# Autodesk Inventor assembly: Assembly1
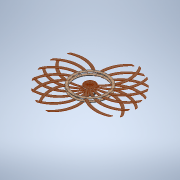
[picture p0: Inventor's stored thumbnail of the model, 180x180]
Saved by Autodesk Inventor 2020.3 (Build 243373000, 373)
## iProperties
Created: 2020-11-01
Part Number: Assembly1
Document SubType Name: Assembly
Designer: Martijn
Author: Martijn
## Documents named in this file (28)
- D:\Documents\GitHub\electrokinetic-sculpture\cad files\Assembly1.iam
- D:\Documents\GitHub\electrokinetic-sculpture\cad files\as.ipt
- D:\Documents\GitHub\electrokinetic-sculpture\cad files\pulley1.ipt
- D:\Documents\GitHub\electrokinetic-sculpture\cad files\wall_mount.ipt
- D:\Documents\GitHub\electrokinetic-sculpture\cad files\GT2 60 teeth pulley.ipt
- D:\Documents\GitHub\electrokinetic-sculpture\cad files\Nema 17 - Busheng 17HD34008-22B\Nema 17 Stepper Motor.iam
- D:\Documents\GitHub\electrokinetic-sculpture\cad files\bearing_holder.ipt
- D:\Documents\GitHub\electrokinetic-sculpture\cad files\bearing_holder2.ipt
- D:\Documents\GitHub\electrokinetic-sculpture\cad files\enclosure.ipt
- D:\Documents\GitHub\electrokinetic-sculpture\cad files\Lock Collar 8mm.ipt
- D:\Documents\GitHub\electrokinetic-sculpture\cad files\spoke.ipt
- D:\Documents\GitHub\electrokinetic-sculpture\cad files\spoke2.ipt
- D:\Documents\GitHub\electrokinetic-sculpture\cad files\cover.ipt
- D:\Documents\GitHub\electrokinetic-sculpture\cad files\pololu-universal-aluminum-mounting-hub-for-8mm-shaft-m3-holes.ipt
- D:\Documents\GitHub\electrokinetic-sculpture\cad files\wheel2.ipt
- D:\Documents\GitHub\electrokinetic-sculpture\cad files\front_plate.ipt
- D:\Documents\GitHub\electrokinetic-sculpture\cad files\spoke3.ipt
- D:\Documents\GitHub\electrokinetic-sculpture\cad files\cover2.ipt
- D:\Documents\GitHub\electrokinetic-sculpture\cad files\wheel3.ipt
- D:\Documents\GitHub\electrokinetic-sculpture\cad files\wheel4.ipt
- D:\Documents\GitHub\electrokinetic-sculpture\cad files\spoke4.ipt
- D:\Documents\GitHub\electrokinetic-sculpture\cad files\wheel5.ipt
- D:\Documents\GitHub\electrokinetic-sculpture\cad files\wheel6.ipt
- D:\Documents\GitHub\electrokinetic-sculpture\cad files\wheel7.ipt
- D:\Documents\GitHub\electrokinetic-sculpture\cad files\wheel8.ipt
- D:\Documents\GitHub\electrokinetic-sculpture\cad files\center_cover.ipt
- D:\Documents\GitHub\electrokinetic-sculpture\cad files\motor_spacer.ipt
- D:\Documents\GitHub\electrokinetic-sculpture\cad files\pulley_bearing_combo.ipt
## Components (72 placed, 27 different names)
1. as:1 — Mate:2, Flush:1, Mate:13, Mate:20, Mate:64, Mate:213, Mate:260, Mate:262, Mate:264
2. pulley1:1 — Mate:22, Mate:24, Mate:27, Mate:30, Mate:33, Mate:61, Mate:63, Mate:66, Mate:212, Mate:213, Mate:214, Mate:215, Mate:216, Mate:217, Mate:218, Mate:219, Mate:220, Mate:221, Mate:222, Mate:223, Mate:224, Mate:225, Mate:226, Mate:227, Mate:228, Mate:229, Mate:230, Mate:231, Mate:232, Mate:233, Mate:234, Mate:235, Mate:236, Mate:237, Mate:238, Mate:239, Mate:240, Mate:241, Mate:242, Mate:244, Mate:245, Mate:246, Mate:247, Mate:248, Mate:249, Mate:250, Mate:251, Mate:252, Mate:253, Mate:254, Mate:255, Mate:256, Mate:257, Mate:258, Mate:259, Mate:261, Mate:266
3. wall_mount:1 — Mate:2, Flush:1, Mate:10, Mate:11, Mate:12, Mate:14, Mate:19, Mate:158, Mate:168
4. Nema 17 Stepper Motor:1 [sub-assembly] — Angle:2, Mate:160, Mate:161, Mate:162
5. bearing_holder:1 — Mate:263, Mate:264, Mate:265
6. bearing_holder2:1 — Mate:10, Mate:11, Mate:12, Mate:21
7. enclosure:1 — Mate:13, Mate:14, Mate:163, Mate:164, Mate:214
8. Nema 17 Stepper Motor:2 [sub-assembly] — Angle:2, Mate:165, Mate:166, Mate:167
9. GT2 60 teeth pulley:1 — Mate:19
10. Lock Collar 8mm:1 — Mate:20, Mate:21
11. spoke:1 — Mate:22, Mate:68, Mate:102, Mate:224, Mate:225
12. spoke:2 — Mate:24, Mate:222, Mate:223
13. spoke:3 — Mate:27, Mate:220, Mate:221
14. spoke:4 — Mate:30, Mate:217, Mate:218
15. spoke:5 — Mate:33, Mate:215, Mate:216, Mate:243
16. spoke2:1 — Mate:51, Mate:54, Mate:74
17. spoke:6 — Mate:66, Mate:67, Mate:219
18. spoke2:2 — Mate:50, Mate:72, Mate:157
19. spoke2:3 — Mate:50, Mate:51, Mate:73
20. spoke2:4 — Mate:54, Mate:57, Mate:75
21. spoke2:5 — Mate:57, Mate:60, Mate:76
22. spoke2:6 — Mate:60, Mate:65, Mate:77
23. cover:1 — Mate:61, Mate:63, Mate:67, Mate:80, Mate:226
24. pololu-universal-aluminum-mounting-hub-for-8mm-shaft-m3-holes:1 — Mate:64, Mate:78
25. wheel2:1 — Mate:65, Mate:69, Flush:2, Mate:70, Mate:72, Mate:73, Mate:74, Mate:75, Mate:76, Mate:77, Mate:135, Mate:136, Mate:137, Mate:138, Mate:157
26. wheel2:2 — Mate:68, Mate:69, Flush:2, Mate:70, Mate:102, Mate:133, Mate:134, Mate:243
27. front_plate:1 — Mate:78, Mate:80, Mate:81, Mate:82, Mate:83, Mate:85, Mate:86, Mate:88, Mate:91, Mate:92, Mate:93, Mate:95, Mate:96, Mate:98, Mate:99, Mate:100, Mate:106, Mate:139, Mate:141, Mate:173, Mate:174, Mate:175, Mate:176, Mate:177, Mate:178, Mate:179, Mate:181, Mate:182, Mate:183, Mate:184, Mate:185, Mate:186, Mate:187, Mate:188, Mate:189, Mate:190, Mate:191, Mate:192, Mate:193, Mate:194, Mate:195, Mate:196, Mate:197, Mate:198, Mate:199, Mate:200, Mate:201, Mate:202, Mate:203, Mate:204, Mate:205, Mate:206, Mate:207, Mate:208, Mate:209, Mate:210, Mate:211, Mate:260
28. spoke3:1 — Mate:81, Mate:82, Mate:172, Mate:178
29. spoke3:2 — Mate:83, Mate:85, Mate:177
30. spoke3:3 — Mate:93, Mate:95, Mate:174
31. spoke3:4 — Mate:86, Mate:88, Mate:169, Mate:170, Mate:171, Mate:176
32. spoke3:5 — Mate:91, Mate:92, Mate:175
33. spoke3:6 — Mate:96, Mate:98, Mate:173
34. cover2:1 — Mate:99, Mate:100, Mate:172, Mate:180
35. wheel3:1 — Mate:106, Flush:3, Mate:108, Mate:109, Mate:127, Mate:130, Mate:131, Mate:132, Mate:169, Mate:170
36. wheel4:1 — Flush:3, Mate:108, Mate:109, Mate:110, Mate:111, Mate:112, Mate:113, Mate:114, Mate:115, Mate:116, Mate:117, Mate:118, Mate:119, Mate:120, Mate:121, Mate:122, Mate:123, Mate:124, Mate:125, Mate:126, Mate:128, Mate:129, Mate:142
37. spoke4:1 — Mate:110, Mate:111, Mate:142
38. spoke4:2 — Mate:112, Mate:113, Mate:114
39. spoke4:3 — Mate:124, Mate:125, Mate:126
40. spoke4:4 — Mate:118, Mate:119, Mate:120
41. spoke4:5 — Mate:115, Mate:116, Mate:117
42. spoke4:6 — Mate:121, Mate:122, Mate:123
43. wheel5:1 — Mate:127, Mate:128, Mate:129
44. wheel6:1 — Mate:130, Mate:131, Mate:132
45. wheel7:1 — Mate:133, Mate:134, Mate:135
46. wheel8:1 — Mate:136, Mate:137, Mate:138
47. center_cover:1 — Mate:139, Mate:141, Mate:171
48. motor_spacer:1 — Mate:158, Mate:160, Mate:161, Mate:162, Mate:168
49. motor_spacer:2 — Mate:163, Mate:164, Mate:165, Mate:166, Mate:167
50. cover2:2 — Mate:179, Mate:180, Mate:181
51. cover2:3 — Mate:182, Mate:183, Mate:184
52. cover2:4 — Mate:191, Mate:193, Mate:194
53. cover2:5 — Mate:188, Mate:189, Mate:190
54. cover2:6 — Mate:192, Mate:195, Mate:196
55. cover2:7 — Mate:185, Mate:186, Mate:187
56. cover2:8 — Mate:206, Mate:207, Mate:208
57. cover2:9 — Mate:199, Mate:202, Mate:203
58. cover2:10 — Mate:197, Mate:204, Mate:205
59. cover2:11 — Mate:198, Mate:200, Mate:201
60. cover2:12 — Mate:209, Mate:210, Mate:211
61. cover:2 — Mate:212, Mate:227, Mate:228
62. cover:4 — Mate:233, Mate:248, Mate:249
63. cover:5 — Mate:230, Mate:252, Mate:253
64. cover:6 — Mate:236, Mate:246, Mate:247
65. cover:7 — Mate:234, Mate:237, Mate:238
66. cover:8 — Mate:235, Mate:244, Mate:245
67. cover:9 — Mate:231, Mate:241, Mate:242
68. cover:10 — Mate:229, Mate:239, Mate:240
69. cover:11 — Mate:232, Mate:250, Mate:251
70. cover:12 — Mate:254, Mate:256, Mate:257
71. cover:13 — Mate:255, Mate:258, Mate:259
72. pulley_bearing_combo:1 — Mate:261, Mate:262, Mate:263, Mate:265, Mate:266
## Relationships (199: Mate 195, Flush 3, Angle 1)
- Mate:2: as:1 ↔ wall_mount:1
- Flush:1: as:1 ↔ wall_mount:1
- Mate:10: wall_mount:1 ↔ bearing_holder2:1
- Mate:11: wall_mount:1 ↔ bearing_holder2:1
- Mate:12: wall_mount:1 ↔ bearing_holder2:1
- Mate:13: as:1 ↔ enclosure:1
- Mate:14: wall_mount:1 ↔ enclosure:1
- Mate:19: wall_mount:1 ↔ GT2 60 teeth pulley:1
- Mate:20: as:1 ↔ Lock Collar 8mm:1
- Mate:21 (7 mm): bearing_holder2:1 ↔ Lock Collar 8mm:1
- Mate:22: pulley1:1 ↔ spoke:1
- Mate:24: pulley1:1 ↔ spoke:2
- Mate:27: pulley1:1 ↔ spoke:3
- Mate:30: pulley1:1 ↔ spoke:4
- Mate:33: pulley1:1 ↔ spoke:5
- Mate:50: spoke2:2 ↔ spoke2:3
- Mate:51: spoke2:1 ↔ spoke2:3
- Mate:54: spoke2:1 ↔ spoke2:4
- Mate:57: spoke2:4 ↔ spoke2:5
- Mate:60: spoke2:5 ↔ spoke2:6
- Mate:61: pulley1:1 ↔ cover:1
- Mate:63: pulley1:1 ↔ cover:1
- Mate:64: as:1 ↔ pololu-universal-aluminum-mounting-hub-for-8mm-shaft-m3-holes:1
- Mate:65: spoke2:6 ↔ wheel2:1
- Mate:66: pulley1:1 ↔ spoke:6
- Mate:67: spoke:6 ↔ cover:1
- Mate:68: spoke:1 ↔ wheel2:2
- Mate:69: wheel2:1 ↔ wheel2:2
- Flush:2: wheel2:1 ↔ wheel2:2
- Mate:70: wheel2:1 ↔ wheel2:2
- Mate:72: spoke2:2 ↔ wheel2:1
- Mate:73: spoke2:3 ↔ wheel2:1
- Mate:74: spoke2:1 ↔ wheel2:1
- Mate:75: spoke2:4 ↔ wheel2:1
- Mate:76: spoke2:5 ↔ wheel2:1
- Mate:77: spoke2:6 ↔ wheel2:1
- Mate:78: pololu-universal-aluminum-mounting-hub-for-8mm-shaft-m3-holes:1 ↔ front_plate:1
- Mate:80 (33 mm): cover:1 ↔ front_plate:1
- Mate:81: front_plate:1 ↔ spoke3:1
- Mate:82: front_plate:1 ↔ spoke3:1
- Mate:83: front_plate:1 ↔ spoke3:2
- Mate:85: front_plate:1 ↔ spoke3:2
- Mate:86: front_plate:1 ↔ spoke3:4
- Mate:88: front_plate:1 ↔ spoke3:4
- Mate:91: front_plate:1 ↔ spoke3:5
- Mate:92: front_plate:1 ↔ spoke3:5
- Mate:93: front_plate:1 ↔ spoke3:3
- Mate:95: front_plate:1 ↔ spoke3:3
- Mate:96: front_plate:1 ↔ spoke3:6
- Mate:98: front_plate:1 ↔ spoke3:6
- Mate:99: front_plate:1 ↔ cover2:1
- Mate:100: front_plate:1 ↔ cover2:1
- Mate:102: spoke:1 ↔ wheel2:2
- Mate:106: front_plate:1 ↔ wheel3:1
- Flush:3: wheel3:1 ↔ wheel4:1
- Mate:108: wheel3:1 ↔ wheel4:1
- Mate:109: wheel3:1 ↔ wheel4:1
- Mate:110: wheel4:1 ↔ spoke4:1
- Mate:111: wheel4:1 ↔ spoke4:1
- Mate:112: wheel4:1 ↔ spoke4:2
- Mate:113: wheel4:1 ↔ spoke4:2
- Mate:114: wheel4:1 ↔ spoke4:2
- Mate:115: wheel4:1 ↔ spoke4:5
- Mate:116: wheel4:1 ↔ spoke4:5
- Mate:117: wheel4:1 ↔ spoke4:5
- Mate:118: wheel4:1 ↔ spoke4:4
- Mate:119: wheel4:1 ↔ spoke4:4
- Mate:120: wheel4:1 ↔ spoke4:4
- Mate:121: wheel4:1 ↔ spoke4:6
- Mate:122: wheel4:1 ↔ spoke4:6
- Mate:123: wheel4:1 ↔ spoke4:6
- Mate:124: wheel4:1 ↔ spoke4:3
- Mate:125: wheel4:1 ↔ spoke4:3
- Mate:126: wheel4:1 ↔ spoke4:3
- Mate:127: wheel3:1 ↔ wheel5:1
- Mate:128: wheel4:1 ↔ wheel5:1
- Mate:129: wheel4:1 ↔ wheel5:1
- Mate:130: wheel3:1 ↔ wheel6:1
- Mate:131: wheel3:1 ↔ wheel6:1
- Mate:132: wheel3:1 ↔ wheel6:1
- Mate:133: wheel2:2 ↔ wheel7:1
- Mate:134: wheel2:2 ↔ wheel7:1
- Mate:135: wheel2:1 ↔ wheel7:1
- Mate:136: wheel2:1 ↔ wheel8:1
- Mate:137: wheel2:1 ↔ wheel8:1
- Mate:138: wheel2:1 ↔ wheel8:1
- Angle:2 (0 deg): Nema 17 Stepper Motor:1 ↔ Nema 17 Stepper Motor:2
- Mate:139: front_plate:1 ↔ center_cover:1
- Mate:141: front_plate:1 ↔ center_cover:1
- Mate:142: wheel4:1 ↔ spoke4:1
- Mate:157: spoke2:2 ↔ wheel2:1
- Mate:158: wall_mount:1 ↔ motor_spacer:1
- Mate:160: Nema 17 Stepper Motor:1 ↔ motor_spacer:1
- Mate:161: Nema 17 Stepper Motor:1 ↔ motor_spacer:1
- Mate:162: Nema 17 Stepper Motor:1 ↔ motor_spacer:1
- Mate:163: enclosure:1 ↔ motor_spacer:2
- Mate:164 (-3.9 mm): enclosure:1 ↔ motor_spacer:2
- Mate:165: Nema 17 Stepper Motor:2 ↔ motor_spacer:2
- Mate:166: Nema 17 Stepper Motor:2 ↔ motor_spacer:2
- Mate:167: Nema 17 Stepper Motor:2 ↔ motor_spacer:2
- Mate:168 (-3.9 mm): wall_mount:1 ↔ motor_spacer:1
- Mate:169: spoke3:4 ↔ wheel3:1
- Mate:170: spoke3:4 ↔ wheel3:1
- Mate:171: spoke3:4 ↔ center_cover:1
- Mate:172: spoke3:1 ↔ cover2:1
- Mate:173: front_plate:1 ↔ spoke3:6
- Mate:174: front_plate:1 ↔ spoke3:3
- Mate:175: front_plate:1 ↔ spoke3:5
- Mate:176: front_plate:1 ↔ spoke3:4
- Mate:177: front_plate:1 ↔ spoke3:2
- Mate:178: front_plate:1 ↔ spoke3:1
- Mate:179: front_plate:1 ↔ cover2:2
- Mate:180: cover2:1 ↔ cover2:2
- Mate:181: front_plate:1 ↔ cover2:2
- Mate:182: front_plate:1 ↔ cover2:3
- Mate:183: front_plate:1 ↔ cover2:3
- Mate:184: front_plate:1 ↔ cover2:3
- Mate:185: front_plate:1 ↔ cover2:7
- Mate:186: front_plate:1 ↔ cover2:7
- Mate:187: front_plate:1 ↔ cover2:7
- Mate:188: front_plate:1 ↔ cover2:5
- Mate:189: front_plate:1 ↔ cover2:5
- Mate:190: front_plate:1 ↔ cover2:5
- Mate:191: front_plate:1 ↔ cover2:4
- Mate:192: front_plate:1 ↔ cover2:6
- Mate:193: front_plate:1 ↔ cover2:4
- Mate:194: front_plate:1 ↔ cover2:4
- Mate:195: front_plate:1 ↔ cover2:6
- Mate:196: front_plate:1 ↔ cover2:6
- Mate:197: front_plate:1 ↔ cover2:10
- Mate:198: front_plate:1 ↔ cover2:11
- Mate:199: front_plate:1 ↔ cover2:9
- Mate:200: front_plate:1 ↔ cover2:11
- Mate:201: front_plate:1 ↔ cover2:11
- Mate:202: front_plate:1 ↔ cover2:9
- Mate:203: front_plate:1 ↔ cover2:9
- Mate:204: front_plate:1 ↔ cover2:10
- Mate:205: front_plate:1 ↔ cover2:10
- Mate:206: front_plate:1 ↔ cover2:8
- Mate:207: front_plate:1 ↔ cover2:8
- Mate:208: front_plate:1 ↔ cover2:8
- Mate:209: front_plate:1 ↔ cover2:12
- Mate:210: front_plate:1 ↔ cover2:12
- Mate:211: front_plate:1 ↔ cover2:12
- Mate:212: pulley1:1 ↔ cover:2
- Mate:213: as:1 ↔ pulley1:1
- Mate:214 (5 mm): pulley1:1 ↔ enclosure:1
- Mate:215: pulley1:1 ↔ spoke:5
- Mate:216: pulley1:1 ↔ spoke:5
- Mate:217: pulley1:1 ↔ spoke:4
- Mate:218: pulley1:1 ↔ spoke:4
- Mate:219: pulley1:1 ↔ spoke:6
- Mate:220: pulley1:1 ↔ spoke:3
- Mate:221: pulley1:1 ↔ spoke:3
- Mate:222: pulley1:1 ↔ spoke:2
- Mate:223: pulley1:1 ↔ spoke:2
- Mate:224: pulley1:1 ↔ spoke:1
- Mate:225: pulley1:1 ↔ spoke:1
- Mate:226: pulley1:1 ↔ cover:1
- Mate:227: pulley1:1 ↔ cover:2
- Mate:228: pulley1:1 ↔ cover:2
- Mate:229: pulley1:1 ↔ cover:10
- Mate:230: pulley1:1 ↔ cover:5
- Mate:231: pulley1:1 ↔ cover:9
- Mate:232: pulley1:1 ↔ cover:11
- Mate:233: pulley1:1 ↔ cover:4
- Mate:234: pulley1:1 ↔ cover:7
- Mate:235: pulley1:1 ↔ cover:8
- Mate:236: pulley1:1 ↔ cover:6
- Mate:237: pulley1:1 ↔ cover:7
- Mate:238: pulley1:1 ↔ cover:7
- Mate:239: pulley1:1 ↔ cover:10
- Mate:240: pulley1:1 ↔ cover:10
- Mate:241: pulley1:1 ↔ cover:9
- Mate:242: pulley1:1 ↔ cover:9
- Mate:243: spoke:5 ↔ wheel2:2
- Mate:244: pulley1:1 ↔ cover:8
- Mate:245: pulley1:1 ↔ cover:8
- Mate:246: pulley1:1 ↔ cover:6
- Mate:247: pulley1:1 ↔ cover:6
- Mate:248: pulley1:1 ↔ cover:4
- Mate:249: pulley1:1 ↔ cover:4
- Mate:250: pulley1:1 ↔ cover:11
- Mate:251: pulley1:1 ↔ cover:11
- Mate:252: pulley1:1 ↔ cover:5
- Mate:253: pulley1:1 ↔ cover:5
- Mate:254: pulley1:1 ↔ cover:12
- Mate:255: pulley1:1 ↔ cover:13
- Mate:256: pulley1:1 ↔ cover:12
- Mate:257: pulley1:1 ↔ cover:12
- Mate:258: pulley1:1 ↔ cover:13
- Mate:259: pulley1:1 ↔ cover:13
- Mate:260: as:1 ↔ front_plate:1
- Mate:261: pulley1:1 ↔ pulley_bearing_combo:1
- Mate:262: as:1 ↔ pulley_bearing_combo:1
- Mate:263: bearing_holder:1 ↔ pulley_bearing_combo:1
- Mate:264: as:1 ↔ bearing_holder:1
- Mate:265: bearing_holder:1 ↔ pulley_bearing_combo:1
- Mate:266: pulley1:1 ↔ pulley_bearing_combo:1
